# Autodesk Inventor assembly: sparAssembly
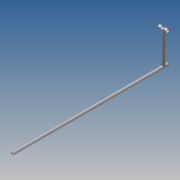
[picture p0: Inventor's stored thumbnail of the model, 180x180]
Saved by Autodesk Inventor 2013 SP2 (Build 170200200, 200)
## iProperties
Created: 2013-12-03
Part Number: sparAssembly
Document SubType Name: Assembly
Designer: Dave
Author: Dave
## Documents named in this file (5)
- C:\Users\Dave\Desktop\hera-cad\support\sparAssembly.iam
- C:\Users\Dave\Desktop\hera-cad\support\sparHoriz.ipt
- C:\Users\Dave\Desktop\hera-cad\smallParts\pvc_T_2in.ipt
- C:\Users\Dave\Desktop\hera-cad\support\sparVert.ipt
- C:\Users\Dave\Desktop\hera-cad\smallParts\pvc_T_2in_modPipe.ipt
## Components (4 placed, 4 different names)
1. sparHoriz:1 — Insert:1
2. pvc_T_2in:1 — Insert:1, Insert:2
3. sparVert:1 — Insert:2, Insert:3
4. pvc_T_2in_modPipe:1 — Insert:3
## Relationships (3: Insert 3)
- Insert:1 (-25.4 mm): sparHoriz:1 ↔ pvc_T_2in:1
- Insert:2 (-25.4 mm): pvc_T_2in:1 ↔ sparVert:1
- Insert:3 (-25.4 mm): sparVert:1 ↔ pvc_T_2in_modPipe:1
